# Autodesk Inventor assembly: Controller_V1
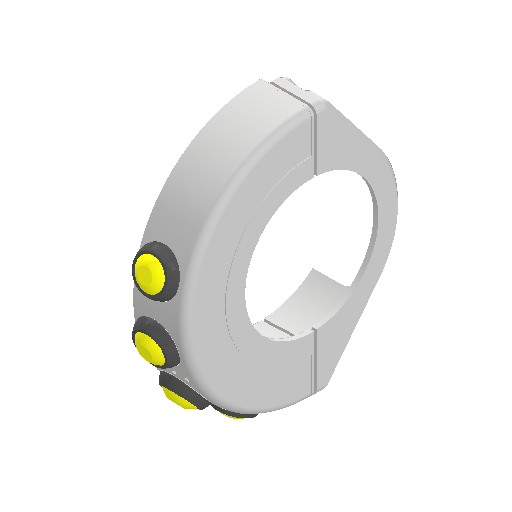
[picture p0: Inventor's stored thumbnail of the model, 512x512]
Saved by Autodesk Inventor 2025.2 (Build 292293000, 293)
## iProperties
Created: 2025-04-17
Part Number: Controller_V1
Document SubType Name: Assembly
Designer: Andreas
Author: Andreas
## Documents named in this file (8)
- C:\Daten\Temp\AdventureController\cad\Controller_V1.iam
- C:\Daten\Temp\AdventureController\cad\nrf52840.ipt
- C:\Daten\Temp\AdventureController\cad\UpperPartFront.ipt
- C:\Daten\Temp\AdventureController\cad\Button_RS_14mm_yellow\Button_RS_14mm_yellow.iam
- C:\Daten\Temp\AdventureController\cad\UperPartBack.ipt
- C:\Daten\Temp\AdventureController\cad\LowerPart.ipt
- C:\Daten\Temp\AdventureController\cad\Nut.ipt
- C:\Daten\Temp\AdventureController\cad\Distance_Piece.ipt
## Components (13 placed, 7 different names)
1. UpperPartFront:1 — Insert:1, Mate:1, Flush:1, Flush:2, Flush:3, Tangent:1, Tangent:2, Mate:2, Mate:3, Mate:5, Mate:8
2. nrf52840:1 — Mate:1, Tangent:1, Tangent:2
3. UperPartBack:1 — Mate:2, Mate:3, Mate:5, Mate:6, Flush:4, Angle:1
4. LowerPart:1 — Mate:6, Flush:4, Angle:1, Mate:9
5. Distance_Piece:1 — Mate:9
6. Button_RS_14mm_yellow:1 [sub-assembly] — Insert:1, Mate:7
7. Nut:1 — Mate:7, Mate:8
8. Button_RS_14mm_yellow:2 [sub-assembly]
9. Nut:2
10. Button_RS_14mm_yellow:3 [sub-assembly]
11. Nut:3
12. Button_RS_14mm_yellow:4 [sub-assembly]
13. Nut:4
## Component patterns: (4 elements, first: Button_RS_14mm_yellow:1 + Nut:1)
## Relationships (16: Mate 8, Flush 4, Tangent 2, Insert 1, Angle 1)
- Insert:1: UpperPartFront:1 ↔ Button_RS_14mm_yellow:1
- Mate:1: UpperPartFront:1 ↔ nrf52840:1
- Flush:1: UpperPartFront:1
- Flush:2: UpperPartFront:1
- Flush:3: UpperPartFront:1
- Tangent:1 (-6 mm): UpperPartFront:1 ↔ nrf52840:1
- Tangent:2 (-2 mm): UpperPartFront:1 ↔ nrf52840:1
- Mate:2: UpperPartFront:1 ↔ UperPartBack:1
- Mate:3: UpperPartFront:1 ↔ UperPartBack:1
- Mate:5: UpperPartFront:1 ↔ UperPartBack:1
- Mate:6: UperPartBack:1 ↔ LowerPart:1
- Flush:4: UperPartBack:1 ↔ LowerPart:1
- Angle:1 (180 deg): UperPartBack:1 ↔ LowerPart:1
- Mate:7: Button_RS_14mm_yellow:1 ↔ Nut:1
- Mate:8: UpperPartFront:1 ↔ Nut:1
- Mate:9: LowerPart:1 ↔ Distance_Piece:1
